# Autodesk Inventor assembly: 組合1
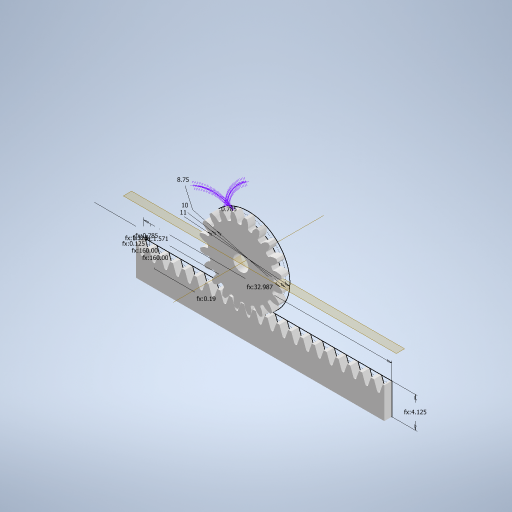
[picture p0: Inventor's stored thumbnail of the model, 512x512]
Saved by Autodesk Inventor 2024 (Build 280153000, 153)
## iProperties
Created: 2024-04-20
Part Number: 組合1
Document SubType Name: Assembly
Designer: rumse
Author: rumse
## Documents named in this file (3)
- C:\文件\機電系統實驗\Electromechanical-System-Principles\抬升機構.iam
- C:\文件\機電系統實驗\Electromechanical-System-Principles\齒條.ipt
- C:\文件\機電系統實驗\Electromechanical-System-Principles\齒輪.ipt
## Components (2 placed, 2 different names)
1. 齒輪:1 — 貼合:1, 相切:1, 貼合:2, 貼合:3, 齊平:1, 貼合:4, 旋轉/轉換:1
2. 齒條:1 — 相切:1, 貼合:2, 齊平:1, 貼合:4, 旋轉/轉換:1, 角度:1
## Relationships (8: Mate 4, Tangent 1, Flush 1, RelateRotateTranslate 1, Angle 1)
- 貼合:1 [Mate]: 齒輪:1
- 相切:1 [Tangent]: 齒輪:1 ↔ 齒條:1
- 貼合:2 [Mate]: 齒輪:1 ↔ 齒條:1
- 貼合:3 [Mate]: 齒輪:1
- 齊平:1 [Flush]: 齒輪:1 ↔ 齒條:1
- 貼合:4 [Mate]: 齒輪:1 ↔ 齒條:1
- 旋轉/轉換:1 [RelateRotateTranslate] (31.416 mm): 齒輪:1 ↔ 齒條:1
- 角度:1 [Angle] (0 deg): 齒條:1
